# Autodesk Inventor assembly: Assembly4
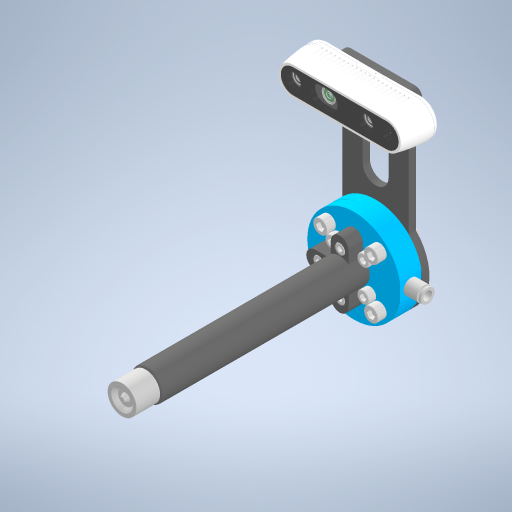
[picture p0: Inventor's stored thumbnail of the model, 512x512]
Saved by Autodesk Inventor 2023 (Build 270158000, 158)
## iProperties
Created: 2022-05-19
Part Number: Assembly4
Document SubType Name: Assembly
Designer: romanp
Author: romanp
## Documents named in this file (13)
- C:\Users\romanp\Downloads\SMC_EE_XT661-2A-R\Assembly_SMC_EE.iam
- C:\Users\romanp\Downloads\SMC_EE_XT661-2A-R\Part_Top_a_Blue.ipt
- C:\Users\romanp\Downloads\SMC_EE_XT661-2A-R\Part_Top_b_Blue.ipt
- C:\Users\romanp\Downloads\SMC_EE_XT661-2A-R\M4x20.ipt
- C:\Users\romanp\Downloads\SMC_EE_XT661-2A-R\M4_nut.ipt
- C:\Users\romanp\Downloads\SMC_EE_XT661-2A-R\IntelRealsense_D435.ipt
- C:\Users\romanp\Downloads\SMC_EE_XT661-2A-R\Part_Type_1_Black.ipt
- C:\Users\romanp\Downloads\SMC_EE_XT661-2A-R\KQ2H06-00A.ipt
- C:\Users\romanp\Downloads\SMC_EE_XT661-2A-R\M5x25.ipt
- C:\Users\romanp\Downloads\SMC_EE_XT661-2A-R\M6x25.ipt
- C:\Users\romanp\Downloads\SMC_EE_XT661-2A-R\Part_Bottom_Black.ipt
- C:\Users\romanp\Downloads\SMC_EE_XT661-2A-R\XT661-2A-R.ipt
- C:\Users\romanp\Downloads\SMC_EE_XT661-2A-R\KQ2H06-M5N.ipt
## Components (22 placed, 12 different names)
1. Part_Top_a_Blue — Insert:1, Insert:9, Insert:10, Insert:21, Insert:22, Insert:23
2. Part_Top_b_Blue — Insert:1, Insert:24, Insert:25, Insert:26, Insert:27, Insert:28, Insert:29, Insert:30, Insert:31, Insert:32, Insert:33
3. M4x20:1
4. IntelRealsense_D435:1 — Insert:11, Insert:12
5. Part_Type_2_Black — Insert:9, Insert:10, Insert:11, Insert:12
6. M4x20:2
7. M4x20:3
8. M4_nut:3 — Insert:22
9. M4_nut:4 — Insert:21
10. M4_nut:5 — Insert:23
11. KQ2H06-00A:1 — Insert:24
12. M5x25:1 — Insert:25
13. M6x25:1 — Insert:26
14. M6x25:2 — Insert:28
15. M6x25:3 — Insert:27
16. M6x25:4 — Insert:29
17. M5x25:2 — Insert:30
18. M5x25:3 — Insert:31
19. M5x25:4 — Insert:32
20. Part_Bottom_Black — Insert:33, Insert:34
21. XT661-2A-R:1 — Insert:34, Insert:35
22. KQ2H06-M5N:1 — Insert:35
## Relationships (20: Insert 20)
- Insert:1: Part_Top_a_Blue ↔ Part_Top_b_Blue
- Insert:9: Part_Top_a_Blue ↔ Part_Type_2_Black
- Insert:10: Part_Top_a_Blue ↔ Part_Type_2_Black
- Insert:11: IntelRealsense_D435:1 ↔ Part_Type_2_Black
- Insert:12: IntelRealsense_D435:1 ↔ Part_Type_2_Black
- Insert:21: Part_Top_a_Blue ↔ M4_nut:4
- Insert:22: Part_Top_a_Blue ↔ M4_nut:3
- Insert:23: Part_Top_a_Blue ↔ M4_nut:5
- Insert:24: Part_Top_b_Blue ↔ KQ2H06-00A:1
- Insert:25: Part_Top_b_Blue ↔ M5x25:1
- Insert:26: Part_Top_b_Blue ↔ M6x25:1
- Insert:27: Part_Top_b_Blue ↔ M6x25:3
- Insert:28: Part_Top_b_Blue ↔ M6x25:2
- Insert:29: Part_Top_b_Blue ↔ M6x25:4
- Insert:30: Part_Top_b_Blue ↔ M5x25:2
- Insert:31: Part_Top_b_Blue ↔ M5x25:3
- Insert:32: Part_Top_b_Blue ↔ M5x25:4
- Insert:33: Part_Top_b_Blue ↔ Part_Bottom_Black
- Insert:34: Part_Bottom_Black ↔ XT661-2A-R:1
- Insert:35: XT661-2A-R:1 ↔ KQ2H06-M5N:1
